# Autodesk Inventor assembly: ASY MSC 500 BELLY
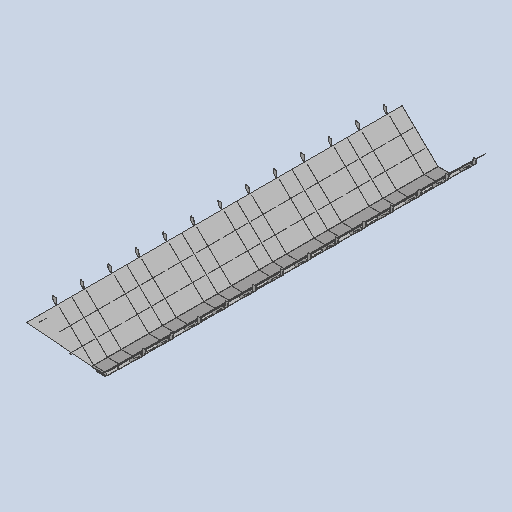
[picture p0: Inventor's stored thumbnail of the model, 512x512]
Saved by Autodesk Inventor 2025 (Build 290162010, 162A)
## iProperties
Created: 2024-07-22
Part Number: ASY MSC 500 BELLY
Document SubType Name: Assembly
Designer: pokla
Stock Number: ASY МОО 500 брюхо
Author: pokla
## Documents named in this file (7)
- C:\Users\DELL\YandexDisk-badmisterfox\домашниий пк\Inventor\Manturovo\Manturovo_Se-clar\ASY MSC 500 BELLY.iam
- C:\Users\DELL\YandexDisk-badmisterfox\домашниий пк\Inventor\Manturovo\Manturovo_Se-clar\MSC 501 sheet belly main.ipt
- C:\Users\DELL\YandexDisk-badmisterfox\домашниий пк\Inventor\Manturovo\Manturovo_Se-clar\MSC 502 sheet belly-neck.ipt
- C:\Users\DELL\YandexDisk-badmisterfox\домашниий пк\Inventor\Manturovo\Manturovo_Se-clar\MSC 504 stringer board belly.ipt
- C:\Users\DELL\YandexDisk-badmisterfox\домашниий пк\Inventor\Manturovo\Manturovo_Se-clar\MSC 503 rib belly.ipt
- C:\Users\DELL\YandexDisk-badmisterfox\домашниий пк\Inventor\Manturovo\Manturovo_Se-clar\MSC 505 STRINGER BOARD BELLY FACE.ipt
- C:\Users\DELL\YandexDisk-badmisterfox\домашниий пк\Inventor\Manturovo\Manturovo_Se-clar\MSC 506 STRINGER BOARD BELLY.ipt
## Components (87 placed, 6 different names)
1. MSC 501 SHEET BELLY MAIN:1
2. MSC 501 SHEET BELLY MAIN:2
3. MSC 501 SHEET BELLY MAIN:3
4. MSC 502 SHEET BELLY-NECK:1 — Rigid:24
5. MSC 501 SHEET BELLY MAIN:4
6. MSC 501 SHEET BELLY MAIN:5 — Rigid:24
7. MSC 501 SHEET BELLY MAIN:6 — Mate:4, Mate:5, Mate:6, Mate:7, Flush:1, Mate:9, Mate:10, Flush:2, Mate:11, Mate:12
8. MSC 503 RIB BELLY:1 — Rigid:17, Rigid:20, Rigid:21, Mate:13, Mate:15, Mate:16, Mate:17
9. MSC 503 RIB BELLY:2 — Rigid:18, Rigid:19, Mate:11, Mate:12, Mate:13, Mate:14, Mate:18, Mate:19
10. MSC 504 STRINGER BOARD BELLY:1 — Rigid:21, Flush:2
11. MSC 504 STRINGER BOARD BELLY:2 — Rigid:20
12. MSC 504 STRINGER BOARD BELLY:3 — Rigid:19
13. MSC 504 STRINGER BOARD BELLY:4 — Rigid:18
14. MSC 505 STRINGER BOARD BELLY FACE:1 — Rigid:25
15. MSC 505 STRINGER BOARD BELLY FACE:2 — Rigid:26
16. MSC 505 STRINGER BOARD BELLY FACE:3
17. MSC 505 STRINGER BOARD BELLY FACE:4 — Rigid:28
18. MSC 506 STRINGER BOARD BELLY:1 — Mate:14, Mate:18, Mate:19, Rigid:29
19. MSC 506 STRINGER BOARD BELLY:2 — Mate:15, Mate:16, Mate:17, Rigid:30
20. MSC 504 STRINGER BOARD BELLY:5
21. MSC 504 STRINGER BOARD BELLY:6
22. MSC 504 STRINGER BOARD BELLY:7
23. MSC 504 STRINGER BOARD BELLY:8
24. MSC 504 STRINGER BOARD BELLY:9
25. MSC 504 STRINGER BOARD BELLY:10
26. MSC 504 STRINGER BOARD BELLY:11
27. MSC 504 STRINGER BOARD BELLY:12
28. MSC 504 STRINGER BOARD BELLY:13
29. MSC 504 STRINGER BOARD BELLY:14
30. MSC 504 STRINGER BOARD BELLY:15
31. MSC 504 STRINGER BOARD BELLY:16
32. MSC 504 STRINGER BOARD BELLY:17
33. MSC 504 STRINGER BOARD BELLY:18
34. MSC 504 STRINGER BOARD BELLY:19
35. MSC 504 STRINGER BOARD BELLY:20
36. MSC 504 STRINGER BOARD BELLY:21 — Rigid:28
37. MSC 504 STRINGER BOARD BELLY:22
38. MSC 504 STRINGER BOARD BELLY:23 — Rigid:25
39. MSC 504 STRINGER BOARD BELLY:24 — Rigid:26
40. MSC 503 RIB BELLY:3 — Mate:6, Mate:7, Mate:8, Rigid:17
41. MSC 503 RIB BELLY:4 — Mate:4, Mate:5, Mate:8
42. MSC 506 STRINGER BOARD BELLY:4 — Rigid:30
43. MSC 506 STRINGER BOARD BELLY:3 — Rigid:29
44. MSC 503 RIB BELLY:5
45. MSC 503 RIB BELLY:6
46. MSC 506 STRINGER BOARD BELLY:5
47. MSC 506 STRINGER BOARD BELLY:16
48. MSC 503 RIB BELLY:7
49. MSC 503 RIB BELLY:8
50. MSC 506 STRINGER BOARD BELLY:6
51. MSC 506 STRINGER BOARD BELLY:17
52. MSC 503 RIB BELLY:9
53. MSC 503 RIB BELLY:10
54. MSC 506 STRINGER BOARD BELLY:7
55. MSC 506 STRINGER BOARD BELLY:18
56. MSC 503 RIB BELLY:11
57. MSC 503 RIB BELLY:12
58. MSC 506 STRINGER BOARD BELLY:8
59. MSC 506 STRINGER BOARD BELLY:19
60. MSC 503 RIB BELLY:13
61. MSC 503 RIB BELLY:14
62. MSC 506 STRINGER BOARD BELLY:9
63. MSC 506 STRINGER BOARD BELLY:20
64. MSC 503 RIB BELLY:15
65. MSC 503 RIB BELLY:16
66. MSC 506 STRINGER BOARD BELLY:10
67. MSC 506 STRINGER BOARD BELLY:21
68. MSC 503 RIB BELLY:17
69. MSC 503 RIB BELLY:18
70. MSC 506 STRINGER BOARD BELLY:11
71. MSC 506 STRINGER BOARD BELLY:22
72. MSC 503 RIB BELLY:19
73. MSC 503 RIB BELLY:20
74. MSC 506 STRINGER BOARD BELLY:12
75. MSC 506 STRINGER BOARD BELLY:23
76. MSC 503 RIB BELLY:21
77. MSC 503 RIB BELLY:22
78. MSC 506 STRINGER BOARD BELLY:13
79. MSC 506 STRINGER BOARD BELLY:24
80. MSC 503 RIB BELLY:23
81. MSC 503 RIB BELLY:24
82. MSC 506 STRINGER BOARD BELLY:14
83. MSC 506 STRINGER BOARD BELLY:25
84. MSC 503 RIB BELLY:25
85. MSC 503 RIB BELLY:26
86. MSC 506 STRINGER BOARD BELLY:15
87. MSC 506 STRINGER BOARD BELLY:26
## Component patterns: (5 elements, first: MSC 504 STRINGER BOARD BELLY:5 + MSC 504 STRINGER BOARD BELLY:6 + MSC 504 STRINGER BOARD BELLY:7 + MSC 504 STRINGER BOARD BELLY:8), (12 elements, first: MSC 503 RIB BELLY:3 + MSC 503 RIB BELLY:4 + MSC 506 STRINGER BOARD BELLY:4 + MSC 506 STRINGER BOARD BELLY:3)
## Relationships (38: WeldJoint 20, Mate 16, Flush 2)
- [WeldJoint]: MSC 501 SHEET BELLY MAIN:1 ↔ MSC 501 SHEET BELLY MAIN:2
- [WeldJoint]: MSC 501 SHEET BELLY MAIN:1 ↔ MSC 501 SHEET BELLY MAIN:3
- [WeldJoint]: MSC 501 SHEET BELLY MAIN:4 ↔ MSC 501 SHEET BELLY MAIN:5
- [WeldJoint]: MSC 501 SHEET BELLY MAIN:3 ↔ MSC 501 SHEET BELLY MAIN:4
- [WeldJoint]: MSC 501 SHEET BELLY MAIN:2 ↔ MSC 501 SHEET BELLY MAIN:6
- [WeldJoint]: MSC 504 STRINGER BOARD BELLY:3 ↔ MSC 504 STRINGER BOARD BELLY:5
- [WeldJoint]: MSC 504 STRINGER BOARD BELLY:4 ↔ MSC 504 STRINGER BOARD BELLY:6
- [WeldJoint]: MSC 504 STRINGER BOARD BELLY:2 ↔ MSC 504 STRINGER BOARD BELLY:7
- [WeldJoint]: MSC 504 STRINGER BOARD BELLY:1 ↔ MSC 504 STRINGER BOARD BELLY:8
- Mate:4: MSC 501 SHEET BELLY MAIN:6 ↔ MSC 503 RIB BELLY:4
- Mate:5: MSC 501 SHEET BELLY MAIN:6 ↔ MSC 503 RIB BELLY:4
- Mate:6: MSC 501 SHEET BELLY MAIN:6 ↔ MSC 503 RIB BELLY:3
- Mate:7: MSC 501 SHEET BELLY MAIN:6 ↔ MSC 503 RIB BELLY:3
- Mate:8: MSC 503 RIB BELLY:3 ↔ MSC 503 RIB BELLY:4
- Flush:1: MSC 501 SHEET BELLY MAIN:6
- Mate:9: MSC 501 SHEET BELLY MAIN:6
- Mate:10: MSC 501 SHEET BELLY MAIN:6
- Rigid:17 [WeldJoint] (490 mm): MSC 503 RIB BELLY:1 ↔ MSC 503 RIB BELLY:3
- Rigid:18 [WeldJoint]: MSC 503 RIB BELLY:2 ↔ MSC 504 STRINGER BOARD BELLY:4
- Rigid:19 [WeldJoint]: MSC 503 RIB BELLY:2 ↔ MSC 504 STRINGER BOARD BELLY:3
- Rigid:20 [WeldJoint]: MSC 503 RIB BELLY:1 ↔ MSC 504 STRINGER BOARD BELLY:2
- Rigid:21 [WeldJoint]: MSC 503 RIB BELLY:1 ↔ MSC 504 STRINGER BOARD BELLY:1
- Flush:2: MSC 501 SHEET BELLY MAIN:6 ↔ MSC 504 STRINGER BOARD BELLY:1
- Mate:11: MSC 501 SHEET BELLY MAIN:6 ↔ MSC 503 RIB BELLY:2
- Mate:12: MSC 501 SHEET BELLY MAIN:6 ↔ MSC 503 RIB BELLY:2
- Mate:13: MSC 503 RIB BELLY:1 ↔ MSC 503 RIB BELLY:2
- Rigid:24 [WeldJoint]: MSC 502 SHEET BELLY-NECK:1 ↔ MSC 501 SHEET BELLY MAIN:5
- Rigid:25 [WeldJoint]: MSC 505 STRINGER BOARD BELLY FACE:1 ↔ MSC 504 STRINGER BOARD BELLY:23
- Rigid:26 [WeldJoint]: MSC 505 STRINGER BOARD BELLY FACE:2 ↔ MSC 504 STRINGER BOARD BELLY:24
- Rigid:28 [WeldJoint]: MSC 505 STRINGER BOARD BELLY FACE:4 ↔ MSC 504 STRINGER BOARD BELLY:21
- Mate:14: MSC 503 RIB BELLY:2 ↔ MSC 506 STRINGER BOARD BELLY:1
- Mate:15: MSC 503 RIB BELLY:1 ↔ MSC 506 STRINGER BOARD BELLY:2
- Mate:16: MSC 503 RIB BELLY:1 ↔ MSC 506 STRINGER BOARD BELLY:2
- Mate:17 (-20 mm): MSC 503 RIB BELLY:1 ↔ MSC 506 STRINGER BOARD BELLY:2
- Mate:18: MSC 503 RIB BELLY:2 ↔ MSC 506 STRINGER BOARD BELLY:1
- Mate:19 (-20 mm): MSC 503 RIB BELLY:2 ↔ MSC 506 STRINGER BOARD BELLY:1
- Rigid:29 [WeldJoint] (-490 mm): MSC 506 STRINGER BOARD BELLY:1 ↔ MSC 506 STRINGER BOARD BELLY:3
- Rigid:30 [WeldJoint] (-490 mm): MSC 506 STRINGER BOARD BELLY:2 ↔ MSC 506 STRINGER BOARD BELLY:4
